# Autodesk Inventor assembly: BATTERIES_CONTROLLER.brd
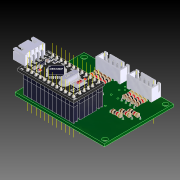
[picture p0: Inventor's stored thumbnail of the model, 180x180]
Saved by Autodesk Inventor 2020 (Build 240168000, 168)
## iProperties
Created: 2021-08-07
Part Number: BATTERIES_CONTROLLER.brd
Document SubType Name: Assembly
Designer: Петров Иван
Mass: 11.1068 g
Surface Area: 165.834 cm^2
Volume: 7.53719 cm^3
Density: 1.4736 g/cm^3
Author: Петров Иван
## Documents named in this file (8)
- E:\IVAN\Ivan_desktop\Kvantorium\Projects\RoboPatrol\electronic\BATTERIES_CONTROLLER\BATTERIES_CONTROLLER.brd.iam
- E:\IVAN\Ivan_desktop\Kvantorium\Projects\RoboPatrol\electronic\BATTERIES_CONTROLLER\BATTERIES_CONTROLLER.brdКонтур.ipt
- E:\IVAN\Ivan_desktop\Kvantorium\Projects\RoboPatrol\design\standart_components\PBS-1.ipt
- E:\IVAN\Ivan_desktop\Kvantorium\Projects\RoboPatrol\design\standart_components\CONN HEADER VERT 1POS 2.54MM.ipt
- E:\IVAN\Ivan_desktop\Kvantorium\Projects\RoboPatrol\design\standart_components\ArduinoProMini\YAAJ_Arduino_ProMini_NanHe.ipt
- E:\IVAN\Ivan_desktop\Kvantorium\Projects\RoboPatrol\design\standart_components\connectrs\JST - XH - Thru (R) - 4Pin - 2.54mm.ipt
- E:\IVAN\Ivan_desktop\Kvantorium\Projects\RoboPatrol\design\standart_components\resistors\1,0 kOhm R Axial DIN0207 L6.3mm D2.5mm P7.62mm Horizontal.ipt
- E:\IVAN\Ivan_desktop\Kvantorium\Projects\RoboPatrol\design\standart_components\connectrs\JST - XH - Thru (V) - 5Pin - 2.54mm.ipt
## Components (75 placed, 7 different names)
1. BATTERIES_CONTROLLER.brdКонтур:1 — Совмещение:1, Совмещение:2, Угол:1, Совмещение:3, Совмещение:4, Совмещение:15, Совмещение:16, Касательность:1, Совмещение:17, Совмещение:18, Касательность:2, Совмещение:19, Совмещение:20, Совмещение:21, Касательность:3, Касательность:4, Касательность:5, Совмещение:22, Совмещение:23, Совмещение:24, Совмещение:25, Совмещение:26, Касательность:6, Совмещение:27, Совмещение:28, Касательность:7, Совмещение:29, Касательность:8, Совмещение:30, Совмещение:31, Совмещение:32, Совмещение:33, Совмещение:34, Совмещение:35
2. YAAJ_Arduino_ProMini_NanHe:1 — Совмещение:9, Совмещение:10, Совмещение:11, Совмещение:12, Совмещение:13, Совмещение:14
3. JST - XH - Thru (R) - 4Pin - 2.54mm:1 — Совмещение:12, Совмещение:13, Совмещение:14
4. 1,0 kOhm R Axial DIN0207 L6.3mm D2.5mm P7.62mm Horizontal:3 — Совмещение:19, Касательность:3, Совмещение:22
5. 1,0 kOhm R Axial DIN0207 L6.3mm D2.5mm P7.62mm Horizontal:4 — Совмещение:20, Касательность:4, Совмещение:23
6. 1,0 kOhm R Axial DIN0207 L6.3mm D2.5mm P7.62mm Horizontal:5 — Совмещение:21, Касательность:5, Совмещение:24
7. 1,0 kOhm R Axial DIN0207 L6.3mm D2.5mm P7.62mm Horizontal:12 — Совмещение:27, Совмещение:28, Касательность:7
8. 1,0 kOhm R Axial DIN0207 L6.3mm D2.5mm P7.62mm Horizontal:13 — Совмещение:29, Касательность:8
9. 1,0 kOhm R Axial DIN0207 L6.3mm D2.5mm P7.62mm Horizontal:14 — Совмещение:25, Совмещение:26, Касательность:6
10. JST - XH - Thru (V) - 5Pin - 2.54mm:1 — Совмещение:30, Совмещение:31, Совмещение:32
11. JST - XH - Thru (V) - 5Pin - 2.54mm:2 — Совмещение:33, Совмещение:34, Совмещение:35
12. PBS-1:3 — Совмещение:1, Совмещение:2, Угол:1, Совмещение:5, Совмещение:6, Заподлицо:1
13. PBS-1:4
14. PBS-1:5
15. PBS-1:6
16. PBS-1:7
17. PBS-1:8
18. PBS-1:9
19. PBS-1:10
20. PBS-1:11
21. PBS-1:12
22. PBS-1:13
23. PBS-1:14
24. PBS-1:15
25. PBS-1:16
26. PBS-1:17
27. PBS-1:18
28. PBS-1:19
29. PBS-1:20
30. PBS-1:21
31. PBS-1:22
32. PBS-1:23
33. PBS-1:24
34. PBS-1:25 — Угол:2
35. PBS-1:26
36. PBS-1:1 — Совмещение:3, Угол:2, Совмещение:4, Совмещение:7, Совмещение:8, Заподлицо:2
37. PBS-1:27
38. PBS-1:28
39. PBS-1:29
40. CONN HEADER VERT 1POS 2.54MM:2 — Совмещение:5, Совмещение:6, Заподлицо:1
41. CONN HEADER VERT 1POS 2.54MM:3
42. CONN HEADER VERT 1POS 2.54MM:4
43. CONN HEADER VERT 1POS 2.54MM:5
44. CONN HEADER VERT 1POS 2.54MM:6
45. CONN HEADER VERT 1POS 2.54MM:7
46. CONN HEADER VERT 1POS 2.54MM:8
47. CONN HEADER VERT 1POS 2.54MM:9
48. CONN HEADER VERT 1POS 2.54MM:10
49. CONN HEADER VERT 1POS 2.54MM:11
50. CONN HEADER VERT 1POS 2.54MM:12
51. CONN HEADER VERT 1POS 2.54MM:13
52. CONN HEADER VERT 1POS 2.54MM:14
53. CONN HEADER VERT 1POS 2.54MM:15
54. CONN HEADER VERT 1POS 2.54MM:16
55. CONN HEADER VERT 1POS 2.54MM:17
56. CONN HEADER VERT 1POS 2.54MM:18
57. CONN HEADER VERT 1POS 2.54MM:19
58. CONN HEADER VERT 1POS 2.54MM:20
59. CONN HEADER VERT 1POS 2.54MM:21
60. CONN HEADER VERT 1POS 2.54MM:22
61. CONN HEADER VERT 1POS 2.54MM:23
62. CONN HEADER VERT 1POS 2.54MM:24 — Совмещение:10
63. CONN HEADER VERT 1POS 2.54MM:25 — Совмещение:9, Совмещение:11
64. CONN HEADER VERT 1POS 2.54MM:1 — Совмещение:7, Совмещение:8, Заподлицо:2
65. CONN HEADER VERT 1POS 2.54MM:26
66. CONN HEADER VERT 1POS 2.54MM:27
67. CONN HEADER VERT 1POS 2.54MM:28
68. 1,0 kOhm R Axial DIN0207 L6.3mm D2.5mm P7.62mm Horizontal:2 — Совмещение:15, Совмещение:16, Касательность:1
69. 1,0 kOhm R Axial DIN0207 L6.3mm D2.5mm P7.62mm Horizontal:6
70. 1,0 kOhm R Axial DIN0207 L6.3mm D2.5mm P7.62mm Horizontal:7
71. 1,0 kOhm R Axial DIN0207 L6.3mm D2.5mm P7.62mm Horizontal:8
72. 1,0 kOhm R Axial DIN0207 L6.3mm D2.5mm P7.62mm Horizontal:1 — Совмещение:17, Совмещение:18, Касательность:2
73. 1,0 kOhm R Axial DIN0207 L6.3mm D2.5mm P7.62mm Horizontal:9
74. 1,0 kOhm R Axial DIN0207 L6.3mm D2.5mm P7.62mm Horizontal:10
75. 1,0 kOhm R Axial DIN0207 L6.3mm D2.5mm P7.62mm Horizontal:11
## Component patterns: (24 elements, first: PBS-1:3), (4 elements, first: PBS-1:1), (24 elements, first: CONN HEADER VERT 1POS 2.54MM:2), (4 elements, first: CONN HEADER VERT 1POS 2.54MM:1), (4 elements, first: 1,0 kOhm R Axial DIN0207 L6.3mm D2.5mm P7.62mm Horizontal:2), (4 elements, first: 1,0 kOhm R Axial DIN0207 L6.3mm D2.5mm P7.62mm Horizontal:1)
## Relationships (47: Mate 35, Tangent 8, Angle 2, Flush 2)
- Совмещение:1 [Mate]: BATTERIES_CONTROLLER.brdКонтур:1 ↔ PBS-1:3
- Совмещение:2 [Mate]: BATTERIES_CONTROLLER.brdКонтур:1 ↔ PBS-1:3
- Угол:1 [Angle] (0 deg): BATTERIES_CONTROLLER.brdКонтур:1 ↔ PBS-1:3
- Совмещение:3 [Mate]: BATTERIES_CONTROLLER.brdКонтур:1 ↔ PBS-1:1
- Угол:2 [Angle] (0 deg): PBS-1:25 ↔ PBS-1:1
- Совмещение:4 [Mate]: BATTERIES_CONTROLLER.brdКонтур:1 ↔ PBS-1:1
- Совмещение:5 [Mate]: PBS-1:3 ↔ CONN HEADER VERT 1POS 2.54MM:2
- Совмещение:6 [Mate]: PBS-1:3 ↔ CONN HEADER VERT 1POS 2.54MM:2
- Заподлицо:1 [Flush]: PBS-1:3 ↔ CONN HEADER VERT 1POS 2.54MM:2
- Совмещение:7 [Mate]: PBS-1:1 ↔ CONN HEADER VERT 1POS 2.54MM:1
- Совмещение:8 [Mate]: PBS-1:1 ↔ CONN HEADER VERT 1POS 2.54MM:1
- Заподлицо:2 [Flush]: PBS-1:1 ↔ CONN HEADER VERT 1POS 2.54MM:1
- Совмещение:9 [Mate]: YAAJ_Arduino_ProMini_NanHe:1 ↔ CONN HEADER VERT 1POS 2.54MM:25
- Совмещение:10 [Mate]: YAAJ_Arduino_ProMini_NanHe:1 ↔ CONN HEADER VERT 1POS 2.54MM:24
- Совмещение:11 [Mate]: YAAJ_Arduino_ProMini_NanHe:1 ↔ CONN HEADER VERT 1POS 2.54MM:25
- Совмещение:12 [Mate]: YAAJ_Arduino_ProMini_NanHe:1 ↔ JST - XH - Thru (R) - 4Pin - 2.54mm:1
- Совмещение:13 [Mate]: YAAJ_Arduino_ProMini_NanHe:1 ↔ JST - XH - Thru (R) - 4Pin - 2.54mm:1
- Совмещение:14 [Mate]: YAAJ_Arduino_ProMini_NanHe:1 ↔ JST - XH - Thru (R) - 4Pin - 2.54mm:1
- Совмещение:15 [Mate]: BATTERIES_CONTROLLER.brdКонтур:1 ↔ 1,0 kOhm R Axial DIN0207 L6.3mm D2.5mm P7.62mm Horizontal:2
- Совмещение:16 [Mate]: BATTERIES_CONTROLLER.brdКонтур:1 ↔ 1,0 kOhm R Axial DIN0207 L6.3mm D2.5mm P7.62mm Horizontal:2
- Касательность:1 [Tangent]: BATTERIES_CONTROLLER.brdКонтур:1 ↔ 1,0 kOhm R Axial DIN0207 L6.3mm D2.5mm P7.62mm Horizontal:2
- Совмещение:17 [Mate]: BATTERIES_CONTROLLER.brdКонтур:1 ↔ 1,0 kOhm R Axial DIN0207 L6.3mm D2.5mm P7.62mm Horizontal:1
- Совмещение:18 [Mate]: BATTERIES_CONTROLLER.brdКонтур:1 ↔ 1,0 kOhm R Axial DIN0207 L6.3mm D2.5mm P7.62mm Horizontal:1
- Касательность:2 [Tangent]: BATTERIES_CONTROLLER.brdКонтур:1 ↔ 1,0 kOhm R Axial DIN0207 L6.3mm D2.5mm P7.62mm Horizontal:1
- Совмещение:19 [Mate]: BATTERIES_CONTROLLER.brdКонтур:1 ↔ 1,0 kOhm R Axial DIN0207 L6.3mm D2.5mm P7.62mm Horizontal:3
- Совмещение:20 [Mate]: BATTERIES_CONTROLLER.brdКонтур:1 ↔ 1,0 kOhm R Axial DIN0207 L6.3mm D2.5mm P7.62mm Horizontal:4
- Совмещение:21 [Mate]: BATTERIES_CONTROLLER.brdКонтур:1 ↔ 1,0 kOhm R Axial DIN0207 L6.3mm D2.5mm P7.62mm Horizontal:5
- Касательность:3 [Tangent]: BATTERIES_CONTROLLER.brdКонтур:1 ↔ 1,0 kOhm R Axial DIN0207 L6.3mm D2.5mm P7.62mm Horizontal:3
- Касательность:4 [Tangent]: BATTERIES_CONTROLLER.brdКонтур:1 ↔ 1,0 kOhm R Axial DIN0207 L6.3mm D2.5mm P7.62mm Horizontal:4
- Касательность:5 [Tangent]: BATTERIES_CONTROLLER.brdКонтур:1 ↔ 1,0 kOhm R Axial DIN0207 L6.3mm D2.5mm P7.62mm Horizontal:5
- Совмещение:22 [Mate]: BATTERIES_CONTROLLER.brdКонтур:1 ↔ 1,0 kOhm R Axial DIN0207 L6.3mm D2.5mm P7.62mm Horizontal:3
- Совмещение:23 [Mate]: BATTERIES_CONTROLLER.brdКонтур:1 ↔ 1,0 kOhm R Axial DIN0207 L6.3mm D2.5mm P7.62mm Horizontal:4
- Совмещение:24 [Mate]: BATTERIES_CONTROLLER.brdКонтур:1 ↔ 1,0 kOhm R Axial DIN0207 L6.3mm D2.5mm P7.62mm Horizontal:5
- Совмещение:25 [Mate]: BATTERIES_CONTROLLER.brdКонтур:1 ↔ 1,0 kOhm R Axial DIN0207 L6.3mm D2.5mm P7.62mm Horizontal:14
- Совмещение:26 [Mate]: BATTERIES_CONTROLLER.brdКонтур:1 ↔ 1,0 kOhm R Axial DIN0207 L6.3mm D2.5mm P7.62mm Horizontal:14
- Касательность:6 [Tangent]: BATTERIES_CONTROLLER.brdКонтур:1 ↔ 1,0 kOhm R Axial DIN0207 L6.3mm D2.5mm P7.62mm Horizontal:14
- Совмещение:27 [Mate]: BATTERIES_CONTROLLER.brdКонтур:1 ↔ 1,0 kOhm R Axial DIN0207 L6.3mm D2.5mm P7.62mm Horizontal:12
- Совмещение:28 [Mate]: BATTERIES_CONTROLLER.brdКонтур:1 ↔ 1,0 kOhm R Axial DIN0207 L6.3mm D2.5mm P7.62mm Horizontal:12
- Касательность:7 [Tangent]: BATTERIES_CONTROLLER.brdКонтур:1 ↔ 1,0 kOhm R Axial DIN0207 L6.3mm D2.5mm P7.62mm Horizontal:12
- Совмещение:29 [Mate]: BATTERIES_CONTROLLER.brdКонтур:1 ↔ 1,0 kOhm R Axial DIN0207 L6.3mm D2.5mm P7.62mm Horizontal:13
- Касательность:8 [Tangent]: BATTERIES_CONTROLLER.brdКонтур:1 ↔ 1,0 kOhm R Axial DIN0207 L6.3mm D2.5mm P7.62mm Horizontal:13
- Совмещение:30 [Mate]: BATTERIES_CONTROLLER.brdКонтур:1 ↔ JST - XH - Thru (V) - 5Pin - 2.54mm:1
- Совмещение:31 [Mate]: BATTERIES_CONTROLLER.brdКонтур:1 ↔ JST - XH - Thru (V) - 5Pin - 2.54mm:1
- Совмещение:32 [Mate]: BATTERIES_CONTROLLER.brdКонтур:1 ↔ JST - XH - Thru (V) - 5Pin - 2.54mm:1
- Совмещение:33 [Mate]: BATTERIES_CONTROLLER.brdКонтур:1 ↔ JST - XH - Thru (V) - 5Pin - 2.54mm:2
- Совмещение:34 [Mate]: BATTERIES_CONTROLLER.brdКонтур:1 ↔ JST - XH - Thru (V) - 5Pin - 2.54mm:2
- Совмещение:35 [Mate]: BATTERIES_CONTROLLER.brdКонтур:1 ↔ JST - XH - Thru (V) - 5Pin - 2.54mm:2
